# Autodesk Inventor assembly: s-assy-gripper_without_finger
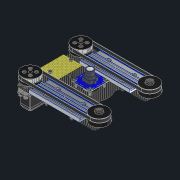
[picture p0: Inventor's stored thumbnail of the model, 180x180]
Saved by Autodesk Inventor 2022 (Build 260153000, 153)
## iProperties
Created: 2021-08-06
Part Number: s-assy-gripper_without_finger
Document SubType Name: Assembly
Designer: yuta0
Mass: 593.374 g
Surface Area: 2184.28 cm^2
Volume: 287.927 cm^3
Density: 2.06085 g/cm^3
Author: yuta0
## Documents named in this file (17)
- C:\Users\yuta0\Documents\GitHub\catchrobo_hardware\assy-scara\s-assy-gripper_without_finger.iam
- C:\Users\yuta0\Documents\GitHub\catchrobo_hardware\assy-scara\carbon_plate14.ipt
- C:\Users\yuta0\Documents\GitHub\catchrobo_hardware\assy-scara\mrs20-100.ipt
- C:\Users\yuta0\Documents\GitHub\catchrobo_hardware\assy-scara\belt4.ipt
- C:\Users\yuta0\Documents\GitHub\catchrobo_hardware\assy-scara\USB Cam model ELP-USBFHD01M-L21.ipt
- C:\Users\yuta0\Documents\GitHub\catchrobo_hardware\assy-scara\CB3-5.ipt
- C:\Users\yuta0\Documents\GitHub\catchrobo_hardware\assy-scara\LBNR4.ipt
- C:\Users\yuta0\Documents\GitHub\catchrobo_hardware\assy-scara\ARU-2010.ipt
- C:\Users\yuta0\Documents\GitHub\catchrobo_hardware\assy-scara\CB2-4.ipt
- C:\Users\yuta0\Documents\GitHub\catchrobo_hardware\assy-scara\d_type_board.ipt
- C:\Users\yuta0\Documents\GitHub\catchrobo_hardware\assy-scara\hexagonal_spacer_M3_5mm.ipt
- C:\Users\yuta0\Documents\GitHub\catchrobo_hardware\assy-scara\LBNR3.ipt
- C:\Users\yuta0\Documents\GitHub\catchrobo_hardware\assy-scara\s-assy-rc_servo.iam
- C:\Users\yuta0\Documents\GitHub\catchrobo_hardware\assy-scara\s-assy-gripper_tentioner.iam
- C:\Users\yuta0\Documents\GitHub\catchrobo_hardware\assy-scara\FU650AD5-C6.ipt
- C:\Users\yuta0\Documents\GitHub\catchrobo_hardware\assy-scara\base21.ipt
- C:\Users\yuta0\Documents\GitHub\catchrobo_hardware\assy-scara\CBSTSR4-14.ipt
## Components (51 placed, 16 different names)
1. carbon_plate14:1 — メイト:1, メイト:2, メイト:3, メイト:51, メイト:52, メイト:53, メイト:90, メイト:92, 角度:1, メイト:98, メイト:102, メイト:103, メイト:104, メイト:105, メイト:106, メイト:107, メイト:109, メイト:110, メイト:111, メイト:113, メイト:139, メイト:140, メイト:141, メイト:142, メイト:143, メイト:144, メイト:147, メイト:150, メイト:183, メイト:197, メイト:200, 角度:4, 角度:5, メイト:201, メイト:202, メイト:203, メイト:207, メイト:208
2. s-assy-rc_servo:1 [sub-assembly] — メイト:139, メイト:140, メイト:141, メイト:145, メイト:146
3. s-assy-rc_servo:2 [sub-assembly] — メイト:142, メイト:143, メイト:144, メイト:153, メイト:154
4. s-assy-gripper_tentioner:1 [sub-assembly] — メイト:147, メイト:149
5. USB Cam model ELP-USBFHD01M-L21:1 — メイト:51, メイト:52, メイト:53, メイト:99, メイト:100, メイト:101
6. hexagonal_spacer_M3_5mm:1 — メイト:106, メイト:107, メイト:108, メイト:114
7. LBNR3:1 — メイト:108, メイト:109
8. LBNR3:2 — メイト:112, メイト:113
9. hexagonal_spacer_M3_5mm:2 — メイト:110, メイト:111, メイト:112
10. d_type_board:1 — メイト:104, メイト:105, メイト:114, メイト:115, メイト:116, メイト:117, メイト:118
11. CB3-5:11 — メイト:115, メイト:116
12. CB3-5:12 — メイト:117, メイト:118
13. belt4:1 — メイト:145, メイト:146, メイト:149
14. belt4:2 — メイト:152, メイト:153, メイト:154
15. FU650AD5-C6:1 — メイト:197, メイト:198, 角度:5
16. FU650AD5-C6:2 — メイト:199, メイト:200, 角度:4
17. base21:1 — メイト:201, メイト:202, メイト:203, メイト:204, メイト:205
18. base21:2 — メイト:206, メイト:207, メイト:208, メイト:209, メイト:210
19. s-assy-gripper_tentioner:2 [sub-assembly] — メイト:150, メイト:152
20. ARU-2010:1 — メイト:98, メイト:99
21. CB2-4:1 — メイト:100, メイト:101
22. CB2-4:2 — メイト:102, メイト:103
23. ARU-2010:2
24. CB2-4:3
25. CB2-4:6
26. ARU-2010:3
27. CB2-4:4
28. CB2-4:7
29. ARU-2010:4
30. CB2-4:5
31. CB2-4:8
32. mrs20-100:2 — メイト:183, メイト:198
33. CBSTSR4-14:2
34. CBSTSR4-14:1
35. LBNR4:4 — メイト:204
36. LBNR4:3 — メイト:205
37. mrs20-100:3
38. CBSTSR4-14:5
39. CBSTSR4-14:6
40. LBNR4:5
41. LBNR4:6
42. mrs20-100:1 — メイト:1, メイト:2, メイト:3, メイト:199
43. CBSTSR4-14:3
44. CBSTSR4-14:4 — メイト:206
45. LBNR4:2 — メイト:92, 角度:1, 角度:2, メイト:209
46. LBNR4:1 — メイト:90, 角度:2, メイト:210
47. mrs20-100:4
48. CBSTSR4-14:7
49. CBSTSR4-14:8
50. LBNR4:7
51. LBNR4:8
## Component patterns: (4 elements, first: ARU-2010:1 + CB2-4:1 + CB2-4:2), (2 elements, first: mrs20-100:2 + CBSTSR4-14:2 + CBSTSR4-14:1 + LBNR4:4 + LBNR4:3), (2 elements, first: mrs20-100:1 + CBSTSR4-14:3 + CBSTSR4-14:4 + LBNR4:2 + LBNR4:1)
## Relationships (75: Mate 70, Angle 5)
- メイト:1 [Mate]: carbon_plate14:1 ↔ mrs20-100:1
- メイト:2 [Mate]: carbon_plate14:1 ↔ mrs20-100:1
- メイト:3 [Mate]: carbon_plate14:1 ↔ mrs20-100:1
- メイト:51 [Mate] (10 mm): carbon_plate14:1 ↔ USB Cam model ELP-USBFHD01M-L21:1
- メイト:52 [Mate]: carbon_plate14:1 ↔ USB Cam model ELP-USBFHD01M-L21:1
- メイト:53 [Mate]: carbon_plate14:1 ↔ USB Cam model ELP-USBFHD01M-L21:1
- メイト:90 [Mate]: carbon_plate14:1 ↔ LBNR4:1
- メイト:92 [Mate]: carbon_plate14:1 ↔ LBNR4:2
- 角度:1 [Angle] (0 deg): carbon_plate14:1 ↔ LBNR4:2
- 角度:2 [Angle] (0 deg): LBNR4:2 ↔ LBNR4:1
- メイト:98 [Mate]: carbon_plate14:1 ↔ ARU-2010:1
- メイト:99 [Mate]: USB Cam model ELP-USBFHD01M-L21:1 ↔ ARU-2010:1
- メイト:100 [Mate]: USB Cam model ELP-USBFHD01M-L21:1 ↔ CB2-4:1
- メイト:101 [Mate]: USB Cam model ELP-USBFHD01M-L21:1 ↔ CB2-4:1
- メイト:102 [Mate]: carbon_plate14:1 ↔ CB2-4:2
- メイト:103 [Mate]: carbon_plate14:1 ↔ CB2-4:2
- メイト:104 [Mate]: carbon_plate14:1 ↔ d_type_board:1
- メイト:105 [Mate]: carbon_plate14:1 ↔ d_type_board:1
- メイト:106 [Mate]: carbon_plate14:1 ↔ hexagonal_spacer_M3_5mm:1
- メイト:107 [Mate]: carbon_plate14:1 ↔ hexagonal_spacer_M3_5mm:1
- メイト:108 [Mate]: hexagonal_spacer_M3_5mm:1 ↔ LBNR3:1
- メイト:109 [Mate]: carbon_plate14:1 ↔ LBNR3:1
- メイト:110 [Mate]: carbon_plate14:1 ↔ hexagonal_spacer_M3_5mm:2
- メイト:111 [Mate]: carbon_plate14:1 ↔ hexagonal_spacer_M3_5mm:2
- メイト:112 [Mate]: LBNR3:2 ↔ hexagonal_spacer_M3_5mm:2
- メイト:113 [Mate]: carbon_plate14:1 ↔ LBNR3:2
- メイト:114 [Mate]: hexagonal_spacer_M3_5mm:1 ↔ d_type_board:1
- メイト:115 [Mate]: d_type_board:1 ↔ CB3-5:11
- メイト:116 [Mate]: d_type_board:1 ↔ CB3-5:11
- メイト:117 [Mate]: d_type_board:1 ↔ CB3-5:12
- メイト:118 [Mate]: d_type_board:1 ↔ CB3-5:12
- [Mate]: mrs20-100:1 ↔ CBSTSR4-14:3
- [Mate]: mrs20-100:1 ↔ CBSTSR4-14:3
- [Mate]: mrs20-100:1 ↔ CBSTSR4-14:4
- [Mate]: mrs20-100:1 ↔ CBSTSR4-14:4
- メイト:139 [Mate]: carbon_plate14:1 ↔ s-assy-rc_servo:1
- メイト:140 [Mate]: carbon_plate14:1 ↔ s-assy-rc_servo:1
- メイト:141 [Mate]: carbon_plate14:1 ↔ s-assy-rc_servo:1
- メイト:142 [Mate]: carbon_plate14:1 ↔ s-assy-rc_servo:2
- メイト:143 [Mate]: carbon_plate14:1 ↔ s-assy-rc_servo:2
- メイト:144 [Mate]: carbon_plate14:1 ↔ s-assy-rc_servo:2
- メイト:145 [Mate]: s-assy-rc_servo:1 ↔ belt4:1
- メイト:146 [Mate] (0.5 mm): s-assy-rc_servo:1 ↔ belt4:1
- メイト:147 [Mate]: carbon_plate14:1 ↔ s-assy-gripper_tentioner:1
- メイト:149 [Mate]: s-assy-gripper_tentioner:1 ↔ belt4:1
- メイト:150 [Mate]: carbon_plate14:1 ↔ s-assy-gripper_tentioner:2
- メイト:152 [Mate]: belt4:2 ↔ s-assy-gripper_tentioner:2
- メイト:153 [Mate]: s-assy-rc_servo:2 ↔ belt4:2
- メイト:154 [Mate] (0.5 mm): s-assy-rc_servo:2 ↔ belt4:2
- [Angle] (0 deg): LBNR4:4 ↔ LBNR4:3
- [Mate]: mrs20-100:2 ↔ CBSTSR4-14:2
- [Mate]: mrs20-100:2 ↔ CBSTSR4-14:2
- [Mate]: mrs20-100:2 ↔ CBSTSR4-14:1
- [Mate]: mrs20-100:2 ↔ CBSTSR4-14:1
- [Mate]: carbon_plate14:1 ↔ CBSTSR4-14:2
- [Mate]: carbon_plate14:1 ↔ CBSTSR4-14:1
- メイト:183 [Mate]: carbon_plate14:1 ↔ mrs20-100:2
- [Mate]: CBSTSR4-14:1 ↔ LBNR4:4
- [Mate]: CBSTSR4-14:2 ↔ LBNR4:3
- メイト:197 [Mate]: carbon_plate14:1 ↔ FU650AD5-C6:1
- メイト:198 [Mate]: FU650AD5-C6:1 ↔ mrs20-100:2
- メイト:199 [Mate]: FU650AD5-C6:2 ↔ mrs20-100:1
- メイト:200 [Mate]: carbon_plate14:1 ↔ FU650AD5-C6:2
- 角度:4 [Angle] (0 deg): carbon_plate14:1 ↔ FU650AD5-C6:2
- 角度:5 [Angle] (0 deg): carbon_plate14:1 ↔ FU650AD5-C6:1
- メイト:201 [Mate]: carbon_plate14:1 ↔ base21:1
- メイト:202 [Mate]: carbon_plate14:1 ↔ base21:1
- メイト:203 [Mate]: carbon_plate14:1 ↔ base21:1
- メイト:204 [Mate]: base21:1 ↔ LBNR4:4
- メイト:205 [Mate]: base21:1 ↔ LBNR4:3
- メイト:206 [Mate]: base21:2 ↔ CBSTSR4-14:4
- メイト:207 [Mate]: carbon_plate14:1 ↔ base21:2
- メイト:208 [Mate]: carbon_plate14:1 ↔ base21:2
- メイト:209 [Mate]: base21:2 ↔ LBNR4:2
- メイト:210 [Mate]: base21:2 ↔ LBNR4:1
## Named parameters: d282_d214 = 0 mm, d283_d215 = 0 mm, d284_d216 = 0 mm, d285_d217 = 0 mm, d286_d170 = 0 deg
